# Autodesk Inventor assembly: 足回り
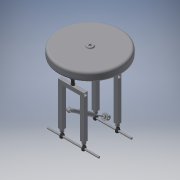
[picture p0: Inventor's stored thumbnail of the model, 180x180]
Saved by Autodesk Inventor 2018 (Build 220112000, 112)
## iProperties
Created: 2017-09-09
Part Number: 足回り
Material: 一般
Document SubType Name: Assembly
Designer: mura5
Author: mura5
## Documents named in this file (7)
- C:\Users\mura5\Documents\RBBR\cart\足回り.iam
- C:\Users\mura5\Documents\RBBR\cart\A.iam
- C:\Users\mura5\Documents\RBBR\cart\前輪.ipt
- C:\Users\mura5\Documents\RBBR\cart\Pipe2.ipt
- C:\Users\mura5\Documents\RBBR\cart\スプリング.iam
- C:\Users\mura5\Documents\RBBR\cart\前輪シャフト.ipt
- C:\Users\mura5\Documents\RBBR\cart\前輪シャフトワッシャー.ipt
## Components (7 placed, 6 different names)
1. 前輪:1 — 回転:1, 回転:2
2. Pipe2:1 — 回転:3
3. スプリング:1 [sub-assembly]
4. 前輪シャフト:1 — 回転:1
5. A:1 [sub-assembly]
6. A:2 [sub-assembly]
7. 前輪シャフトワッシャー:1 — 回転:2, 回転:3
## Relationships (3: RevoluteJoint 3)
- 回転:1 [RevoluteJoint]: 前輪:1 ↔ 前輪シャフト:1
- 回転:2 [RevoluteJoint]: 前輪:1 ↔ 前輪シャフトワッシャー:1
- 回転:3 [RevoluteJoint]: Pipe2:1 ↔ 前輪シャフトワッシャー:1
